# Autodesk Inventor assembly: main
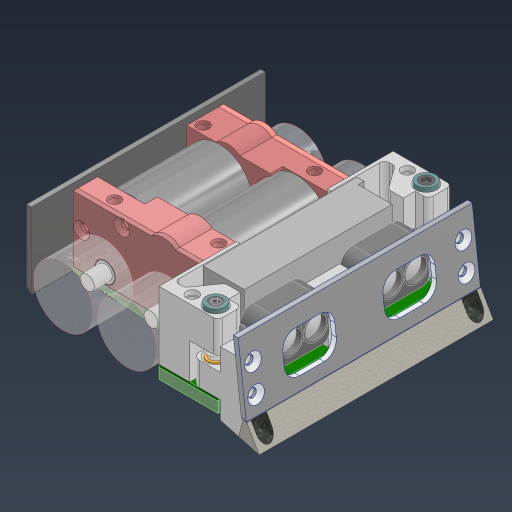
[picture p0: Inventor's stored thumbnail of the model, 512x512]
Saved by Autodesk Inventor 2023 (Build 270158000, 158)
## iProperties
Created: 2025-03-29
Part Number: main
Document SubType Name: Assembly
Designer: szymo
Mass: 469.374 g
Surface Area: 1412.79 cm^2
Volume: 221.065 cm^3
Density: 2.12324 g/cm^3
Author: szymo
## Documents named in this file (23)
- D:\tech\robotyka\robots\evangelion\inventor-project\main rev2.iam
- D:\tech\robotyka\robots\evangelion\inventor-project\base.ipt
- D:\tech\robotyka\robots\evangelion\inventor-project\Sensor LUNA.ipt
- D:\tech\robotyka\robots\evangelion\inventor-project\rs385.ipt
- D:\tech\robotyka\robots\evangelion\inventor-project\back.ipt
- D:\tech\robotyka\robots\evangelion\inventor-project\Gears\Design Accelerator\Przekładnia walcowa13.ipt
- D:\tech\robotyka\robots\evangelion\inventor-project\tattu450_2s.ipt
- D:\tech\robotyka\robots\evangelion\inventor-project\smol-gear-stack.iam
- D:\tech\robotyka\robots\evangelion\inventor-project\big-gear-stack.iam
- D:\tech\robotyka\robots\evangelion\inventor-project\enormous-gear-long.iam
- D:\tech\robotyka\robots\evangelion\inventor-project\enormous-gear-short.iam
- D:\tech\robotyka\robots\evangelion\inventor-project\front.iam
- D:\tech\robotyka\robots\evangelion\inventor-project\right-side-front-mechanism.iam
- D:\tech\robotyka\robots\evangelion\inventor-project\front-lunas-holder.ipt
- D:\tech\robotyka\robots\evangelion\inventor-project\gearbox-holder-right.ipt
- D:\tech\robotyka\robots\evangelion\inventor-project\gearbox-holder-left.ipt
- D:\tech\robotyka\robots\evangelion\inventor-project\right-side-front-mechanism_MIR.iam
- D:\tech\robotyka\robots\evangelion\inventor-project\PCB-dummy.ipt
- D:\tech\robotyka\robots\evangelion\inventor-project\XT30.ipt
- D:\tech\robotyka\robots\evangelion\inventor-project\PCB-INTERFACE-dummy.ipt
- D:\tech\robotyka\robots\evangelion\inventor-project\ceil.ipt
- D:\tech\robotyka\robots\evangelion\inventor-project\gearbox-wall-right.ipt
- D:\tech\robotyka\robots\evangelion\inventor-project\gearbox-wall-left.ipt
## Components (33 placed, 22 different names)
1. base:1 — Tangent:1, Tangent:2, Tangent:3, Mate:1, Mate:2, Angle:4, Mate:17, Flush:3, Angle:7, Tangent:41, Tangent:42, Flush:10, Flush:23, Flush:24, Flush:25, Flush:29, Mate:48, Mate:50, Flush:52, Flush:53, Mate:53, Mate:55, Flush:54, Flush:55, Flush:56, Flush:57, Flush:58, Flush:60, Flush:61, Flush:63, Mate:62, Flush:71, Flush:72
2. back:1 — Mate:17, Flush:3, Tangent:30, Tangent:38, Flush:64, Angle:8, Angle:9, Tangent:55
3. ceil:1 — Flush:64
4. rs385:3 — Tangent:1, Tangent:3, Tangent:4, Mate:2, Tangent:32, Mate:36, Mate:37, Tangent:40, Tangent:42, Tangent:46, Tangent:47, Angle:9, Tangent:55
5. rs385:2 — Tangent:2, Tangent:4, Mate:1, Mate:15, Mate:16, Tangent:41, Tangent:44, Tangent:45, Tangent:52, Tangent:53, Tangent:54, Angle:8
6. Przekładnia walcowa1:5 — Mate:36, Mate:37
7. smol-gear-stack:6 [sub-assembly]
8. smol-gear-stack:5 [sub-assembly] — Tangent:45, Tangent:54
9. big-gear-stack:3 [sub-assembly]
10. enormous-gear-short:2 [sub-assembly] — Tangent:39, Angle:7, Tangent:44, Mate:47
11. enormous-gear-long:4 [sub-assembly] — Tangent:38, Tangent:39, Tangent:40, Mate:46
12. gearbox-holder-left:1 — Flush:29, Flush:70
13. gearbox-wall-left:1 — Flush:70
14. Przekładnia walcowa1:4 — Mate:15, Mate:16
15. smol-gear-stack:3 [sub-assembly] — Tangent:47
16. big-gear-stack:2 [sub-assembly] — Mate:12, Tangent:29, Mate:29
17. smol-gear-stack:4 [sub-assembly]
18. enormous-gear-long:3 [sub-assembly] — Mate:12, Angle:4, Mate:30, Tangent:31, Mate:47
19. enormous-gear-short:1 [sub-assembly] — Tangent:29, Mate:29, Mate:30, Tangent:30, Tangent:31, Tangent:32, Tangent:46, Mate:46, Mate:48, Flush:56, Flush:57
20. gearbox-holder-right:1 — Flush:25, Flush:28, Flush:58, Flush:59, Flush:60, Flush:61, Flush:63, Flush:69
21. gearbox-wall-right:1 — Flush:69
22. right-side-front-mechanism_MIR:1 [sub-assembly] — Mate:56
23. front-lunas-holder:1 — Flush:23, Flush:24
24. front:1 [sub-assembly] — Flush:10
25. right-side-front-mechanism:1 [sub-assembly] — Flush:28, Mate:52
26. PCB-dummy:1 — Mate:62, Flush:71, Flush:72
27. PCB-INTERFACE-dummy:1 — Flush:59
28. Sensor LUNA:2 — Flush:54, Mate:60
29. Sensor LUNA:1 — Flush:55, Mate:61
30. tattu450_2s:1 — Mate:50, Tangent:52, Flush:52, Mate:51, Mate:54, Mate:57, Mate:60, Mate:61
31. tattu450_2s:2 — Mate:51, Tangent:53, Flush:53
32. XT30:1 — Mate:52, Mate:53, Mate:54
33. XT30:3 — Mate:55, Mate:56, Mate:57
## Relationships (95: Mate 32, Tangent 31, Flush 28, Angle 4)
- Tangent:1: base:1 ↔ rs385:3
- Tangent:2: base:1 ↔ rs385:2
- Tangent:3: base:1 ↔ rs385:3
- Tangent:4: rs385:3 ↔ rs385:2
- Mate:1 (25.3 mm): base:1 ↔ rs385:2
- Mate:2 (25.3 mm): base:1 ↔ rs385:3
- [Tangent]: Przekładnia walcowa1:4 ↔ smol-gear-stack:4
- [Flush]: Przekładnia walcowa1:4 ↔ smol-gear-stack:4
- [Tangent]: smol-gear-stack:3 ↔ smol-gear-stack:4
- [Mate] (0.1 mm): smol-gear-stack:3 ↔ smol-gear-stack:4
- [Tangent]: smol-gear-stack:3 ↔ big-gear-stack:2
- [Mate] (0.1 mm): smol-gear-stack:3 ↔ big-gear-stack:2
- [Tangent]: big-gear-stack:2 ↔ enormous-gear-long:3
- Mate:12 (0.1 mm): big-gear-stack:2 ↔ enormous-gear-long:3
- Mate:15: rs385:2 ↔ Przekładnia walcowa1:4
- Angle:4 (0 deg): base:1 ↔ enormous-gear-long:3
- Mate:16 (0.5 mm): rs385:2 ↔ Przekładnia walcowa1:4
- Mate:17: base:1 ↔ back:1
- Flush:3: base:1 ↔ back:1
- Tangent:29: big-gear-stack:2 ↔ enormous-gear-short:1
- Mate:29 (0.1 mm): big-gear-stack:2 ↔ enormous-gear-short:1
- Mate:30: enormous-gear-long:3 ↔ enormous-gear-short:1
- Tangent:30 (1 mm): back:1 ↔ enormous-gear-short:1
- Tangent:31 (2 mm): enormous-gear-long:3 ↔ enormous-gear-short:1
- Tangent:32 (0.2 mm): rs385:3 ↔ enormous-gear-short:1
- [Tangent]: Przekładnia walcowa1:5 ↔ smol-gear-stack:6
- [Flush]: Przekładnia walcowa1:5 ↔ smol-gear-stack:6
- [Tangent]: smol-gear-stack:6 ↔ smol-gear-stack:5
- [Mate] (0.1 mm): smol-gear-stack:6 ↔ smol-gear-stack:5
- [Tangent]: smol-gear-stack:5 ↔ big-gear-stack:3
- [Mate] (0.1 mm): smol-gear-stack:5 ↔ big-gear-stack:3
- [Tangent]: big-gear-stack:3 ↔ enormous-gear-long:4
- [Mate] (0.1 mm): big-gear-stack:3 ↔ enormous-gear-long:4
- [Tangent]: big-gear-stack:3 ↔ enormous-gear-short:2
- [Mate] (0.1 mm): big-gear-stack:3 ↔ enormous-gear-short:2
- [Mate]: enormous-gear-short:2 ↔ enormous-gear-long:4
- Mate:36: rs385:3 ↔ Przekładnia walcowa1:5
- Mate:37 (0.5 mm): rs385:3 ↔ Przekładnia walcowa1:5
- Tangent:38 (1 mm): back:1 ↔ enormous-gear-long:4
- Tangent:39 (2 mm): enormous-gear-short:2 ↔ enormous-gear-long:4
- Tangent:40 (0.1 mm): rs385:3 ↔ enormous-gear-long:4
- Angle:7 (0 deg): base:1 ↔ enormous-gear-short:2
- Tangent:41: base:1 ↔ rs385:2
- Tangent:42: base:1 ↔ rs385:3
- Tangent:44 (1 mm): rs385:2 ↔ enormous-gear-short:2
- Tangent:45 (2 mm): rs385:2 ↔ smol-gear-stack:5
- Tangent:46 (1 mm): rs385:3 ↔ enormous-gear-short:1
- Tangent:47 (1 mm): rs385:3 ↔ smol-gear-stack:3
- Flush:10: base:1 ↔ front:1
- [Mate]: base:1 ↔ right-side-front-mechanism:1
- [Tangent] (3.5 mm): base:1 ↔ right-side-front-mechanism:1
- [Flush]: base:1 ↔ right-side-front-mechanism:1
- [Flush]: base:1 ↔ right-side-front-mechanism:1
- [Flush]: front:1 ↔ right-side-front-mechanism:1
- Flush:23: base:1 ↔ front-lunas-holder:1
- Flush:24: base:1 ↔ front-lunas-holder:1
- Mate:46: enormous-gear-long:4 ↔ enormous-gear-short:1
- Mate:47: enormous-gear-short:2 ↔ enormous-gear-long:3
- Flush:25: base:1 ↔ gearbox-holder-right:1
- Flush:28 (-33.3 mm): gearbox-holder-right:1 ↔ right-side-front-mechanism:1
- Flush:29: base:1 ↔ gearbox-holder-left:1
- Mate:48: base:1 ↔ enormous-gear-short:1
- Mate:50 (1 mm): base:1 ↔ tattu450_2s:1
- Tangent:52 (0.3 mm): rs385:2 ↔ tattu450_2s:1
- Flush:52 (17 mm): base:1 ↔ tattu450_2s:1
- Mate:51: tattu450_2s:1 ↔ tattu450_2s:2
- Tangent:53 (0.3 mm): rs385:2 ↔ tattu450_2s:2
- Flush:53 (17 mm): base:1 ↔ tattu450_2s:2
- Mate:52 (0.5 mm): right-side-front-mechanism:1 ↔ XT30:1
- Mate:53 (1 mm): base:1 ↔ XT30:1
- Mate:54 (1 mm): tattu450_2s:1 ↔ XT30:1
- Mate:55 (1 mm): base:1 ↔ XT30:3
- Mate:56 (0.5 mm): right-side-front-mechanism_MIR:1 ↔ XT30:3
- Mate:57 (1 mm): tattu450_2s:1 ↔ XT30:3
- Flush:54 (15 mm): base:1 ↔ Sensor LUNA:2
- Flush:55 (15 mm): base:1 ↔ Sensor LUNA:1
- Mate:60 (0.3 mm): Sensor LUNA:2 ↔ tattu450_2s:1
- Mate:61 (0.3 mm): Sensor LUNA:1 ↔ tattu450_2s:1
- Flush:56: base:1 ↔ enormous-gear-short:1
- Flush:57: base:1 ↔ enormous-gear-short:1
- Flush:58: base:1 ↔ gearbox-holder-right:1
- Flush:59: gearbox-holder-right:1 ↔ PCB-INTERFACE-dummy:1
- Flush:60: base:1 ↔ gearbox-holder-right:1
- Flush:61: base:1 ↔ gearbox-holder-right:1
- Flush:63: base:1 ↔ gearbox-holder-right:1
- Flush:64: back:1 ↔ ceil:1
- Flush:69: gearbox-holder-right:1 ↔ gearbox-wall-right:1
- Flush:70: gearbox-holder-left:1 ↔ gearbox-wall-left:1
- Mate:62: base:1 ↔ PCB-dummy:1
- Flush:71: base:1 ↔ PCB-dummy:1
- Flush:72: base:1 ↔ PCB-dummy:1
- Tangent:54 (1 mm): rs385:2 ↔ smol-gear-stack:5
- Angle:8 (0 deg): back:1 ↔ rs385:2
- Angle:9 (180 deg): back:1 ↔ rs385:3
- Tangent:55: back:1 ↔ rs385:3
## Named parameters: d399_d384 = 0 mm, d400_d385 = 0.1 mm, d401_d386 = 0 mm, d402_d387 = 0.1 mm, d404_d389 = 0 mm, d405_d390 = 0.1 mm, d408_d378 = 0 mm, d409_d381 = 0 mm, d471_d399_d384 = 0 mm, d472_d400_d385 = 0.1 mm, d473_d401_d386 = 0 mm, d474_d402_d387 = 0.1 mm, d475_d404_d389 = 0 mm, d476_d405_d390 = 0.1 mm, d477_d408_d378 = 0 mm, d478_d409_d381 = 0 mm, d479_d465 = 0 mm, d480_d466 = 0.1 mm, d481_d467 = 0 mm
